# Autodesk Inventor assembly: X_CarriageR_V2_1_Short
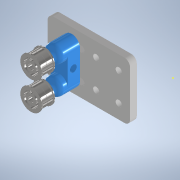
[picture p0: Inventor's stored thumbnail of the model, 180x180]
Saved by Autodesk Inventor 2021 (Build 250183000, 183)
## iProperties
Created: 2021-06-13
Part Number: X_CarriageR_V2_1_Short
Document SubType Name: Assembly
Designer: Jorian Brusind
Author: Jorian Brusind
## Documents named in this file (5)
- C:\Users\Jorian Brusind\Documents\GitHub\HyperRail\Inventor Files\X_CarriageR_V2_1_Short.iam
- C:\Users\Jorian Brusind\Documents\GitHub\HyperRail\Inventor Files\4mm_Roller_Spacer_simple.ipt
- C:\Users\Jorian Brusind\Documents\GitHub\HyperRail\Inventor Files\X_Carriage_Plate_Short.ipt
- C:\Users\Jorian Brusind\Documents\GitHub\HyperRail\Inventor Files\miniature-ball-bearings-metric-series-flanged-1.snapshot.1\F606ZZFlanged\F608 - 8 x 22 x 7.ipt
- C:\Users\Jorian Brusind\Documents\GitHub\PersonalProjects\HyperRail\Inventor Files\miniature-ball-bearings-metric-series-flanged-1.snapshot.1\F606ZZFlanged.ipt
## Components (6 placed, 3 different names)
1. X_Carriage_Plate_Short:1 — Mate:6, Mate:9, Angle:1
2. 4mm_Roller_Spacer_simple:1 — Mate:6, Mate:9, Angle:1, Mate:14, Mate:15, Mate:16, Mate:17
3. F608 - 8 x 22 x 7:4 — Mate:10, Mate:11
4. F608 - 8 x 22 x 7:5 — Mate:10, Mate:11, Mate:14, Mate:15
5. F608 - 8 x 22 x 7:6 — Mate:16
6. F608 - 8 x 22 x 7:7 — Mate:17
## Relationships (11: Mate 10, Angle 1)
- Mate:6: X_Carriage_Plate_Short:1 ↔ 4mm_Roller_Spacer_simple:1
- Mate:9 (-12.5 mm): X_Carriage_Plate_Short:1 ↔ 4mm_Roller_Spacer_simple:1
- Angle:1 (0 deg): X_Carriage_Plate_Short:1 ↔ 4mm_Roller_Spacer_simple:1
- Mate:10: F608 - 8 x 22 x 7:4 ↔ F608 - 8 x 22 x 7:5
- Mate:11: F608 - 8 x 22 x 7:4 ↔ F608 - 8 x 22 x 7:5
- [Mate]: F608 - 8 x 22 x 7:6 ↔ F608 - 8 x 22 x 7:7
- [Mate]: F608 - 8 x 22 x 7:6 ↔ F608 - 8 x 22 x 7:7
- Mate:14: 4mm_Roller_Spacer_simple:1 ↔ F608 - 8 x 22 x 7:5
- Mate:15: 4mm_Roller_Spacer_simple:1 ↔ F608 - 8 x 22 x 7:5
- Mate:16: 4mm_Roller_Spacer_simple:1 ↔ F608 - 8 x 22 x 7:6
- Mate:17: 4mm_Roller_Spacer_simple:1 ↔ F608 - 8 x 22 x 7:7
## Named parameters: d100_d98 = 0 mm, d101_d99 = 0 mm
